# Autodesk Inventor assembly: leg_1
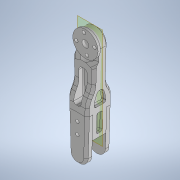
[picture p0: Inventor's stored thumbnail of the model, 180x180]
Saved by Autodesk Inventor 2020 (Build 240168000, 168)
## iProperties
Created: 2019-04-28
Part Number: leg_1
Document SubType Name: Assembly
Designer: psrob
Author: psrob
## Documents named in this file (4)
- E:\projects-2\project dog gen2\hardware\leg_1.iam
- E:\projects-2\project dog gen2\hardware\leg_bone_1.ipt
- E:\projects-2\project dog gen2\hardware\leg_bone_2.ipt
- E:\projects-2\project dog gen2\hardware\flange_6mm.ipt
## Components (4 placed, 3 different names)
1. leg_bone_1:1 — Flush:1, Insert:1, Insert:2, Insert:3, Insert:4, Insert:5
2. leg_bone_2:1 — Flush:1, Insert:1, Insert:2
3. leg_bone_2:2 — Insert:3, Insert:4
4. flange_6mm:1 — Insert:5
## Relationships (6: Insert 5, Flush 1)
- Flush:1: leg_bone_1:1 ↔ leg_bone_2:1
- Insert:1: leg_bone_1:1 ↔ leg_bone_2:1
- Insert:2: leg_bone_1:1 ↔ leg_bone_2:1
- Insert:3: leg_bone_1:1 ↔ leg_bone_2:2
- Insert:4: leg_bone_1:1 ↔ leg_bone_2:2
- Insert:5 (-2 mm): leg_bone_1:1 ↔ flange_6mm:1
